# Autodesk Inventor assembly: CAD Assembly2
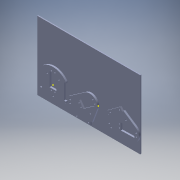
[picture p0: Inventor's stored thumbnail of the model, 180x180]
Saved by Autodesk Inventor 2016 (Build 200138000, 138)
## iProperties
Created: 2018-04-01
Part Number: CAD Assembly2
Document SubType Name: Assembly
Designer: Nuwan
Sending System: SolidWorks 2014
Last Author: Nuwan
Last Saved: 2018-04-02
Author: Nuwan
## Documents named in this file (4)
- D:\Projects\Robot Arm\robort-arm\cad\inventor\CAD Assembly2.iam
- D:\Projects\Robot Arm\robort-arm\cad\inventor\workpiece-base.ipt
- D:\Projects\Robot Arm\robort-arm\cad\inventor\base11.ipt
- D:\Projects\Robot Arm\robort-arm\cad\inventor\base12.ipt
## Components (4 placed, 3 different names)
1. workpiece-base:2 — Mate:1, Mate:2, Mate:4, Flush:1, Mate:5
2. base11:1 — Mate:1
3. base12:1 — Mate:2, Mate:4, Flush:1
4. base12:2 — Mate:5
## Relationships (5: Mate 4, Flush 1)
- Mate:1: workpiece-base:2 ↔ base11:1
- Mate:2: workpiece-base:2 ↔ base12:1
- Mate:4: workpiece-base:2 ↔ base12:1
- Flush:1 (5 mm): workpiece-base:2 ↔ base12:1
- Mate:5: workpiece-base:2 ↔ base12:2
